# Autodesk Inventor assembly: сборка захвата
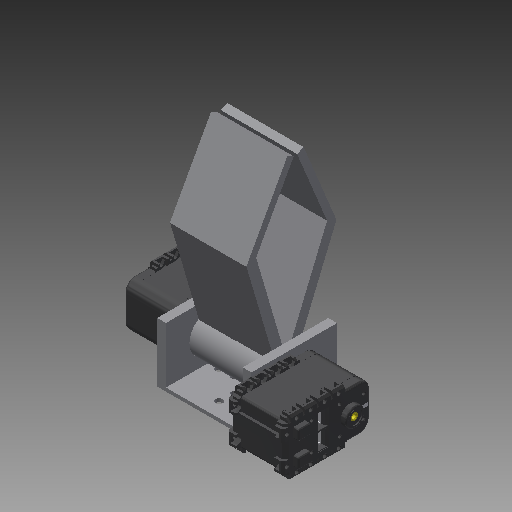
[picture p0: Inventor's stored thumbnail of the model, 512x512]
Saved by Autodesk Inventor 2019 (Build 230136000, 136)
## iProperties
Created: 2019-08-15
Part Number: сборка захвата
Material: Типовые
Document SubType Name: Assembly
Designer: Петров Иван
Author: Петров Иван
## Documents named in this file (4)
- C:\Users\user\Documents\Kvantoriada2019\optimal_gripper\hardware\Стандартные изделия\Концевик механический\клешня\сборка захвата.iam
- C:\Users\user\Documents\Kvantoriada2019\optimal_gripper\hardware\Стандартные изделия\Концевик механический\клешня\база захвата.ipt
- C:\Users\user\Documents\Kvantoriada2019\optimal_gripper\hardware\Стандартные изделия\Сервомотор Dynamixel AX-12A\ax-12a.iam
- C:\Users\user\Documents\Kvantoriada2019\optimal_gripper\hardware\Стандартные изделия\Концевик механический\клешня\палец.ipt
## Components (5 placed, 3 different names)
1. база захвата:1 — Совмещение:1, Совмещение:2, Совмещение:3, Совмещение:4, Совмещение:5, Совмещение:6
2. ax-12a:1 [sub-assembly] — Совмещение:1, Совмещение:2, Совмещение:3, Совмещение:9, Совмещение:10
3. ax-12a:2 [sub-assembly] — Совмещение:4, Совмещение:5, Совмещение:6, Совмещение:7, Совмещение:8
4. палец:1 — Совмещение:7, Совмещение:8, Направление навивки:1
5. палец:2 — Совмещение:9, Совмещение:10, Направление навивки:1
## Relationships (11: Mate 10, RelateRotation 1)
- Совмещение:1 [Mate]: база захвата:1 ↔ ax-12a:1
- Совмещение:2 [Mate]: база захвата:1 ↔ ax-12a:1
- Совмещение:3 [Mate]: база захвата:1 ↔ ax-12a:1
- Совмещение:4 [Mate]: база захвата:1 ↔ ax-12a:2
- Совмещение:5 [Mate]: база захвата:1 ↔ ax-12a:2
- Совмещение:6 [Mate]: база захвата:1 ↔ ax-12a:2
- Совмещение:7 [Mate]: ax-12a:2 ↔ палец:1
- Совмещение:8 [Mate]: ax-12a:2 ↔ палец:1
- Совмещение:9 [Mate]: ax-12a:1 ↔ палец:2
- Совмещение:10 [Mate]: ax-12a:1 ↔ палец:2
- Направление навивки:1 [RelateRotation] (1 ul): палец:1 ↔ палец:2
